# Autodesk Inventor assembly: kaiseki
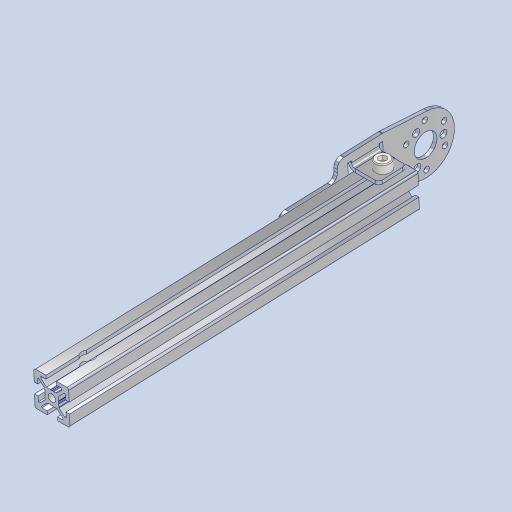
[picture p0: Inventor's stored thumbnail of the model, 512x512]
Saved by Autodesk Inventor 2023 (Build 270158000, 158)
## iProperties
Created: 2024-12-03
Part Number: kaiseki
Document SubType Name: Assembly
Designer: kiyo
Author: kiyo
## Documents named in this file (12)
- D:\GitHub\inventor\syu-si\OfficeRobot\ReadyMade\Aluminum-frame\test\kaiseki.iam
- D:\GitHub\inventor\syu-si\OfficeRobot\ReadyMade\Screw\SCB5-8.ipt
- D:\GitHub\inventor\syu-si\OfficeRobot\Manipulator\pitch_plate_20mm.ipt
- D:\GitHub\inventor\syu-si\OfficeRobot\ReadyMade\Screw\HNTU5-5.ipt
- D:\GitHub\inventor\syu-si\OfficeRobot\ReadyMade\Screw\SCB5-22.ipt
- D:\GitHub\inventor\syu-si\OfficeRobot\ReadyMade\Aluminum-frame\NFS5-2020-200-AV10-BV179.ipt
- D:\GitHub\inventor\syu-si\OfficeRobot\ReadyMade\Aluminum-frame\test\kaiseki\AIP\FEA\ewgmw1xsw.fins
- D:\GitHub\inventor\syu-si\OfficeRobot\ReadyMade\Aluminum-frame\test\kaiseki\AIP\FEA\ewgmw1xsw.fsat
- D:\GitHub\inventor\syu-si\OfficeRobot\ReadyMade\Aluminum-frame\test\kaiseki\AIP\FEA\ewgmw1xsw.ftes
- D:\GitHub\inventor\syu-si\OfficeRobot\ReadyMade\Aluminum-frame\test\kaiseki\AIP\FEA\ewgmw1xsw.fwiz
- D:\GitHub\inventor\syu-si\OfficeRobot\ReadyMade\Aluminum-frame\test\kaiseki\AIP\FEA\ewgmw1xuo.fmsh
- D:\GitHub\inventor\syu-si\OfficeRobot\ReadyMade\Aluminum-frame\test\kaiseki\AIP\FEA\ewgmw1xup.fres
## Components (8 placed, 5 different names)
1. pitch_plate_20mm:1 — メイト:8, 正接:5
2. HNTU5-5:1
3. SCB5-8:2
4. HNTU5-5:2
5. SCB5-22:1
6. NFS5-2020-200-AV10-BV179:1 — メイト:9, 角度:2
7. HNTU5-5:3 — メイト:9, 角度:2
8. SCB5-8:3 — メイト:8, 正接:5
## Relationships (17: Mate 8, Tangent 4, Insert 3, Angle 2)
- [Insert] (3.2 mm): HNTU5-5:1 ↔ SCB5-8:2
- [Angle] (0 deg): pitch_plate_20mm:1 ↔ HNTU5-5:1
- [Tangent] (0.25 mm): pitch_plate_20mm:1 ↔ SCB5-8:2
- [Mate]: pitch_plate_20mm:1 ↔ SCB5-8:2
- [Mate]: pitch_plate_20mm:1 ↔ NFS5-2020-200-AV10-BV179:1
- [Mate]: pitch_plate_20mm:1 ↔ NFS5-2020-200-AV10-BV179:1
- [Mate] (1 mm): HNTU5-5:1 ↔ NFS5-2020-200-AV10-BV179:1
- [Insert] (-0.95 mm): HNTU5-5:2 ↔ SCB5-22:1
- [Mate]: pitch_plate_20mm:1 ↔ SCB5-22:1
- [Tangent] (0.25 mm): pitch_plate_20mm:1 ↔ SCB5-22:1
- [Mate] (1 mm): HNTU5-5:2 ↔ NFS5-2020-200-AV10-BV179:1
- [Tangent] (7.5 mm): SCB5-22:1 ↔ NFS5-2020-200-AV10-BV179:1
- [Insert] (3.2 mm): HNTU5-5:3 ↔ SCB5-8:3
- メイト:8 [Mate]: pitch_plate_20mm:1 ↔ SCB5-8:3
- メイト:9 [Mate] (1 mm): NFS5-2020-200-AV10-BV179:1 ↔ HNTU5-5:3
- 角度:2 [Angle] (0 deg): NFS5-2020-200-AV10-BV179:1 ↔ HNTU5-5:3
- 正接:5 [Tangent] (0.25 mm): pitch_plate_20mm:1 ↔ SCB5-8:3
## Named parameters: d733_d492_d466 = 3.2 mm, d770_d470 = -0.95 mm, d14_d733_d492_d466 = 3.2 mm, sa_0 = 480, sa_1 = 1270, sa_2 = 1270
note: some values were not read from the file. Shown as the stored number, unit unknown: "sa_0", "sa_1", "sa_2".
